# Autodesk Inventor assembly: Chassis, Wheels, and Drive Train Assembly
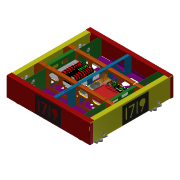
[picture p0: Inventor's stored thumbnail of the model, 180x180]
Saved by Autodesk Inventor 2015 (Build 190159000, 159)
## iProperties
Created: 2015-01-24
Part Number: Chassis, Wheels, and Drive Train Assembly
Document SubType Name: Assembly
Designer: Peter
Author: Peter
## Documents named in this file (6)
- C:\Users\Noah\Desktop\FIRST-Team-1719-CAD-Team\2015 Robot CAD\Chassis, Wheels, and Drive Train\Chassis, Wheels, and Drive Train Assembly.iam
- C:\Users\Noah\Desktop\FIRST-Team-1719-CAD-Team\2015 Robot CAD\Chassis, Wheels, and Drive Train\Chassis - Production Model\Chassis - Production Model.iam
- C:\Users\Noah\Desktop\FIRST-Team-1719-CAD-Team\2015 Robot CAD\Number Plate\Number Plate.ipt
- C:\Users\Noah\Desktop\FIRST-Team-1719-CAD-Team\2015 Robot CAD\Chassis, Wheels, and Drive Train\Mechanum Wheel\Chassis - Wheel.iam
- C:\Users\Noah\Desktop\FIRST-Team-1719-CAD-Team\2015 Robot CAD\Electrical\Electrical Board A.iam
- C:\Users\Noah\Desktop\FIRST-Team-1719-CAD-Team\2015 Robot CAD\Electrical\Electrical Board B.iam
## Components (11 placed, 5 different names)
1. Chassis - Production Model:1 [sub-assembly] — Mate:1, Mate:2, Mate:3, Mate:4, Flush:1, Flush:2, Flush:3, Flush:4, Flush:5, Mate:5, Mate:6, Mate:7, Mate:8, Mate:9, Mate:10, Flush:7, Flush:8, Mate:11, Flush:9, Mate:12, Mate:13, Flush:10, Flush:11, Mate:14, Flush:12, Mate:15
2. Number Plate:1 — Mate:14, Flush:12, Mate:15
3. Number Plate:2 — Mate:10, Flush:7, Flush:8
4. Number Plate:3 — Mate:11, Flush:9, Mate:12
5. Number Plate:4 — Mate:13, Flush:10, Flush:11
6. Chassis - Wheel:1 [sub-assembly] — Mate:3, Flush:1, Flush:4
7. Chassis - Wheel:2 [sub-assembly] — Mate:4, Flush:3
8. Chassis - Wheel:3 [sub-assembly] — Mate:2, Flush:2
9. Chassis - Wheel:4 [sub-assembly] — Mate:1, Flush:5
10. Electrical Board A:1 [sub-assembly] — Mate:5, Flush:6, Mate:7
11. Electrical Board B:1 [sub-assembly] — Mate:6, Flush:6, Mate:8, Mate:9
## Relationships (27: Mate 15, Flush 12)
- Mate:1: Chassis - Production Model:1 ↔ Chassis - Wheel:4
- Mate:2: Chassis - Production Model:1 ↔ Chassis - Wheel:3
- Mate:3: Chassis - Production Model:1 ↔ Chassis - Wheel:1
- Mate:4: Chassis - Production Model:1 ↔ Chassis - Wheel:2
- Flush:1: Chassis - Production Model:1 ↔ Chassis - Wheel:1
- Flush:2: Chassis - Production Model:1 ↔ Chassis - Wheel:3
- Flush:3: Chassis - Production Model:1 ↔ Chassis - Wheel:2
- Flush:4: Chassis - Production Model:1 ↔ Chassis - Wheel:1
- Flush:5: Chassis - Production Model:1 ↔ Chassis - Wheel:4
- Mate:5 (88.9 mm): Chassis - Production Model:1 ↔ Electrical Board A:1
- Mate:6 (88.9 mm): Chassis - Production Model:1 ↔ Electrical Board B:1
- Flush:6: Electrical Board A:1 ↔ Electrical Board B:1
- Mate:7 (8.3185 mm): Chassis - Production Model:1 ↔ Electrical Board A:1
- Mate:8 (8.3185 mm): Chassis - Production Model:1 ↔ Electrical Board B:1
- Mate:9 (5.588 mm): Chassis - Production Model:1 ↔ Electrical Board B:1
- Mate:10: Chassis - Production Model:1 ↔ Number Plate:2
- Flush:7 (12.7 mm): Chassis - Production Model:1 ↔ Number Plate:2
- Flush:8 (234.95 mm): Chassis - Production Model:1 ↔ Number Plate:2
- Mate:11: Chassis - Production Model:1 ↔ Number Plate:3
- Flush:9 (12.7 mm): Chassis - Production Model:1 ↔ Number Plate:3
- Mate:12 (234.95 mm): Chassis - Production Model:1 ↔ Number Plate:3
- Mate:13: Chassis - Production Model:1 ↔ Number Plate:4
- Flush:10 (-12.7 mm): Chassis - Production Model:1 ↔ Number Plate:4
- Flush:11 (234.95 mm): Chassis - Production Model:1 ↔ Number Plate:4
- Mate:14: Chassis - Production Model:1 ↔ Number Plate:1
- Flush:12 (12.7 mm): Chassis - Production Model:1 ↔ Number Plate:1
- Mate:15 (234.95 mm): Chassis - Production Model:1 ↔ Number Plate:1
